# Autodesk Inventor assembly: Assembly1
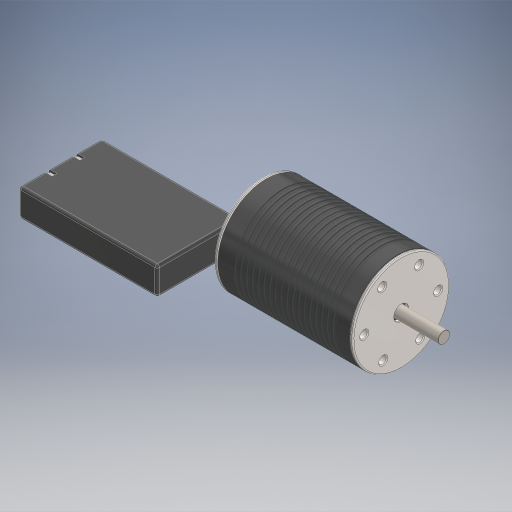
[picture p0: Inventor's stored thumbnail of the model, 512x512]
Saved by Autodesk Inventor 2024 (Build 280153000, 153)
## iProperties
Created: 2024-04-02
Part Number: Assembly1
Document SubType Name: Assembly
Designer: Alex
Author: Alex
## Documents named in this file (3)
- C:\Shared\alex-bartella-schoolwork\4z03\final\Assembly1.iam
- C:\Shared\alex-bartella-schoolwork\4z03\Week 11\STEP files for CE 12.2 & 13.1\rc_battery\rc_battery.ipt
- C:\Shared\alex-bartella-schoolwork\4z03\Week 11\STEP files for CE 12.2 & 13.1\rc_motor\rc_motor.ipt
## Components (2 placed, 2 different names)
1. rc_battery:1
2. rc_motor:1 — Mate:1, Flush:1
## Relationships (2: Mate 1, Flush 1)
- Mate:1: rc_motor:1
- Flush:1: rc_motor:1
